# Autodesk Inventor assembly: Main
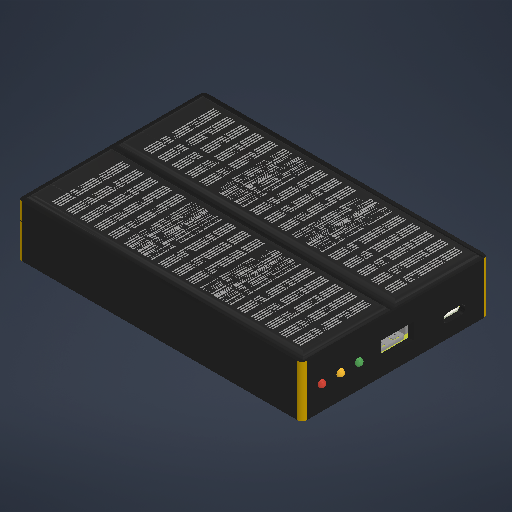
[picture p0: Inventor's stored thumbnail of the model, 512x512]
Saved by Autodesk Inventor 2027.1 (Build 311270010, 270A)
## iProperties
Created: 2026-09-18
Part Number: Main
Document SubType Name: Assembly
Designer: Rozkurwiator
Author: Rozkurwiator
## Documents named in this file (12)
- G:\Github\Solarbank\Hardware\Model\Main.iam
- G:\Github\Solarbank\Hardware\PCB\Power_bank_PCB\PCB\PCB\PCB.ipt
- G:\Github\Solarbank\Hardware\Model\Parts\Battery_prop.ipt
- G:\Github\Solarbank\Hardware\Model\Parts\Bottom.ipt
- G:\Github\Solarbank\Hardware\Model\Parts\led 3 mm amarillo\led 3 mm amarillo.ipt
- G:\Github\Solarbank\Hardware\Model\Parts\OscarML_Led 3mm Rojo v1\OscarML_Led 3mm Rojo v1.ipt
- G:\Github\Solarbank\Hardware\Model\Parts\OscarML_Led 3mm Verde\OscarML_Led 3mm Verde.ipt
- G:\Github\Solarbank\Hardware\Model\Parts\SolarPanel_30x65x3mm\SolarPanel_30x65x3mm.ipt
- G:\Github\Solarbank\Hardware\Model\Parts\Micro_Button_6x6\Micro_Button_6x6.ipt
- G:\Github\Solarbank\Hardware\Model\Parts\Top_part.ipt
- G:\Github\Solarbank\Hardware\Model\Parts\92000A022_Passivated 18-8 Stainless Steel Pan Head Phillips Screws\92000A022_Passivated 18-8 Stainless Steel Pan Head Phillips Screws.ipt
- G:\Github\Solarbank\Hardware\Model\Parts\94459A767_Heat-Set Inserts for Plastic\94459A767_Heat-Set Inserts for Plastic.ipt
## Components (28 placed, 11 different names)
1. PCB:1 — Obrotowe:6
2. Battery_prop:1 — Sztywne:1
3. Bottom:1 — Sztywne:1, Obrotowe:2, Obrotowe:3, Obrotowe:4, Sztywne:2, Sztywne:3, Obrotowe:6, Obrotowe:8
4. led 3 mm amarillo:1 — Obrotowe:3
5. OscarML_Led 3mm Rojo v1:1 — Obrotowe:4
6. OscarML_Led 3mm Verde:1 — Obrotowe:2
7. Micro_Button_6x6:1 — Sztywne:2
8. Top_part:1 — Obrotowe:5, Sztywne:3, Obrotowe:7
9. 94459A767_Heat-Set Inserts for Plastic:1 — Obrotowe:7
10. 94459A767_Heat-Set Inserts for Plastic:2
11. 94459A767_Heat-Set Inserts for Plastic:3
12. 94459A767_Heat-Set Inserts for Plastic:4
13. 92000A022_Passivated 18-8 Stainless Steel Pan Head Phillips Screws:1 — Obrotowe:8
14. 92000A022_Passivated 18-8 Stainless Steel Pan Head Phillips Screws:2
15. 92000A022_Passivated 18-8 Stainless Steel Pan Head Phillips Screws:3
16. 92000A022_Passivated 18-8 Stainless Steel Pan Head Phillips Screws:4
17. SolarPanel_30x65x3mm:1 — Obrotowe:5
18. SolarPanel_30x65x3mm:2
19. SolarPanel_30x65x3mm:3
20. SolarPanel_30x65x3mm:4
21. SolarPanel_30x65x3mm:5
22. SolarPanel_30x65x3mm:6
23. SolarPanel_30x65x3mm:7
24. SolarPanel_30x65x3mm:8
25. SolarPanel_30x65x3mm:9
26. SolarPanel_30x65x3mm:10
27. SolarPanel_30x65x3mm:11
28. SolarPanel_30x65x3mm:12
## Component patterns: (2 elements), (4 elements, first: 94459A767_Heat-Set Inserts for Plastic:1), (4 elements, first: 92000A022_Passivated 18-8 Stainless Steel Pan Head Phillips Screws:1), (6 elements, first: SolarPanel_30x65x3mm:1), Szyk komponentów 1:2 (6 elements)
## Relationships (10: RevoluteJoint 7, WeldJoint 3)
- Sztywne:1 [WeldJoint] (5 mm): Battery_prop:1 ↔ Bottom:1
- Obrotowe:2 [RevoluteJoint]: Bottom:1 ↔ OscarML_Led 3mm Verde:1
- Obrotowe:3 [RevoluteJoint]: Bottom:1 ↔ led 3 mm amarillo:1
- Obrotowe:4 [RevoluteJoint]: Bottom:1 ↔ OscarML_Led 3mm Rojo v1:1
- Sztywne:2 [WeldJoint]: Bottom:1 ↔ Micro_Button_6x6:1
- Obrotowe:5 [RevoluteJoint] (3 mm): Top_part:1 ↔ SolarPanel_30x65x3mm:1
- Sztywne:3 [WeldJoint] (-14 mm): Bottom:1 ↔ Top_part:1
- Obrotowe:6 [RevoluteJoint]: PCB:1 ↔ Bottom:1
- Obrotowe:7 [RevoluteJoint]: Top_part:1 ↔ 94459A767_Heat-Set Inserts for Plastic:1
- Obrotowe:8 [RevoluteJoint]: Bottom:1 ↔ 92000A022_Passivated 18-8 Stainless Steel Pan Head Phillips Screws:1
